# Autodesk Inventor assembly: PCB_Case_Assembly1
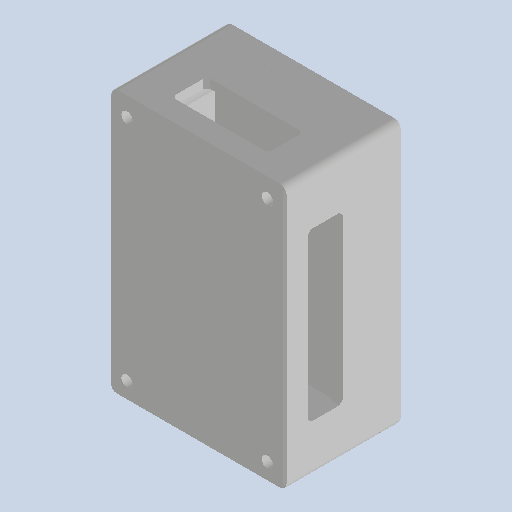
[picture p0: Inventor's stored thumbnail of the model, 512x512]
Saved by Autodesk Inventor 2025.3 (Build 293356000, 356)
## iProperties
Created: 2025-11-23
Part Number: PCB_Case_Assembly1
Document SubType Name: Assembly
Designer: Wula
Author: Wula
## Documents named in this file (4)
- D:\Sabi\gogogo\KIT\Hiwi\WBK_Mikrocontroller\ct_door_opening_sensor\ct_door_opening_sensor\CAD\PCB_Case_Assembly1.iam
- D:\Sabi\gogogo\KIT\Hiwi\WBK_Mikrocontroller\ct_door_opening_sensor\ct_door_opening_sensor\CAD\PCB_Case.ipt
- D:\Sabi\gogogo\KIT\Hiwi\WBK_Mikrocontroller\ct_door_opening_sensor\ct_door_opening_sensor\CAD\PCB_Cover.ipt
- D:\Sabi\gogogo\KIT\Hiwi\WBK_Mikrocontroller\ct_door_opening_sensor\ct_door_opening_sensor\CAD\PCB.ipt
## Components (3 placed, 3 different names)
1. PCB_Case:1 — Mate:2, Mate:3, Mate:4, Flush:1, Flush:2
2. PCB_Cover:1 — Mate:4, Flush:1, Flush:2
3. PCB:1 — Mate:2, Mate:3
## Relationships (5: Mate 3, Flush 2)
- Mate:2: PCB_Case:1 ↔ PCB:1
- Mate:3: PCB_Case:1 ↔ PCB:1
- Mate:4: PCB_Case:1 ↔ PCB_Cover:1
- Flush:1: PCB_Case:1 ↔ PCB_Cover:1
- Flush:2: PCB_Case:1 ↔ PCB_Cover:1
